# Autodesk Inventor assembly: main
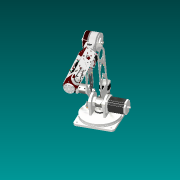
[picture p0: Inventor's stored thumbnail of the model, 180x180]
Saved by Autodesk Inventor 2020.3 (Build 243373000, 373)
## iProperties
Created: 2020-05-24
Part Number: main
Document SubType Name: Assembly
Designer: Svend
Author: Svend
## Documents named in this file (5)
- C:\Users\Svend\OneDrive\Documents\GitHub\BeerMinder\3D-model\mainAssembly\main.iam
- C:\Users\Svend\OneDrive\Documents\GitHub\BeerMinder\3D-model\axis3\axis3.iam
- C:\Users\Svend\OneDrive\Documents\GitHub\BeerMinder\3D-model\Base (Axis 1)\gefreesd\AssemblyGefreesdBasev2.iam
- C:\Users\Svend\OneDrive\Documents\GitHub\BeerMinder\3D-model\axis5_6\axis5_6  compact.iam
- C:\Users\Svend\OneDrive\Documents\GitHub\BeerMinder\3D-model\ControlBox\swithces\Assembly - V-156-1C25 micro switch (Idle).iam
## Components (7 placed, 4 different names)
1. axis3:1 [sub-assembly] — Mate:3, Mate:4, Mate:5, Mate:6, Angle:3, Mate:11, Flush:4, Flush:5, Angle:4, Tangent:1, Flush:6
2. AssemblyGefreesdBasev2:1 [sub-assembly] — Mate:1, Mate:2, Flush:1, Mate:3, Mate:4, Mate:9, Mate:10, Angle:2, Flush:3
3. axis5_6  compact:1 [sub-assembly] — Mate:5, Mate:6
4. Assembly - V-156-1C25 micro switch (Idle):2 [sub-assembly]
5. Assembly - V-156-1C25 micro switch (Idle):1 [sub-assembly] — Mate:9, Mate:10, Angle:2, Flush:3
6. Assembly - V-156-1C25 micro switch (Idle):3 [sub-assembly] — Angle:3, Mate:11, Flush:4, Flush:5
7. Assembly - V-156-1C25 micro switch (Idle):4 [sub-assembly] — Angle:4, Tangent:1, Flush:6
## Relationships (21: Mate 10, Flush 6, Angle 4, Tangent 1)
- Mate:1: AssemblyGefreesdBasev2:1
- Mate:2: AssemblyGefreesdBasev2:1
- Flush:1: AssemblyGefreesdBasev2:1
- Mate:3: axis3:1 ↔ AssemblyGefreesdBasev2:1
- Mate:4: axis3:1 ↔ AssemblyGefreesdBasev2:1
- Mate:5: axis3:1 ↔ axis5_6  compact:1
- Mate:6: axis3:1 ↔ axis5_6  compact:1
- [Mate] (2 mm): AssemblyGefreesdBasev2:1 ↔ Assembly - V-156-1C25 micro switch (Idle):2
- [Angle] (180 deg): AssemblyGefreesdBasev2:1 ↔ Assembly - V-156-1C25 micro switch (Idle):2
- [Flush] (19 mm): AssemblyGefreesdBasev2:1 ↔ Assembly - V-156-1C25 micro switch (Idle):2
- Mate:9 (95 mm): AssemblyGefreesdBasev2:1 ↔ Assembly - V-156-1C25 micro switch (Idle):1
- Mate:10: AssemblyGefreesdBasev2:1 ↔ Assembly - V-156-1C25 micro switch (Idle):1
- Angle:2 (0 deg): AssemblyGefreesdBasev2:1 ↔ Assembly - V-156-1C25 micro switch (Idle):1
- Flush:3 (35 mm): AssemblyGefreesdBasev2:1 ↔ Assembly - V-156-1C25 micro switch (Idle):1
- Angle:3 (180 deg): axis3:1 ↔ Assembly - V-156-1C25 micro switch (Idle):3
- Mate:11: axis3:1 ↔ Assembly - V-156-1C25 micro switch (Idle):3
- Flush:4: axis3:1 ↔ Assembly - V-156-1C25 micro switch (Idle):3
- Flush:5 (-128 mm): axis3:1 ↔ Assembly - V-156-1C25 micro switch (Idle):3
- Angle:4 (210 deg): axis3:1 ↔ Assembly - V-156-1C25 micro switch (Idle):4
- Tangent:1: axis3:1 ↔ Assembly - V-156-1C25 micro switch (Idle):4
- Flush:6: axis3:1 ↔ Assembly - V-156-1C25 micro switch (Idle):4
